# Autodesk Inventor assembly: GripperBaseOnly
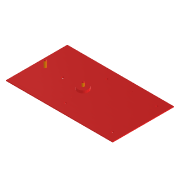
[picture p0: Inventor's stored thumbnail of the model, 180x180]
Saved by Autodesk Inventor 2021 (Build 250183000, 183)
## iProperties
Created: 2022-10-24
Part Number: GripperBaseOnly
Document SubType Name: Assembly
Designer: brian
Author: brian
## Documents named in this file (2)
- G:\Mi unidad\Universidad\Control\Robotica\Laboratorio\Proyecto\Archivos SAT\GripperBasePlace.iam
- G:\Mi unidad\Universidad\Control\Robotica\Laboratorio\Proyecto\GriperBase2.ipt
## Components (1 placed, 1 different names)
1. GriperBase2:1 — Mate:1, Tangent:1, Tangent:2
## Relationships (3: Tangent 2, Mate 1)
- Mate:1: GriperBase2:1
- Tangent:1: GriperBase2:1
- Tangent:2: GriperBase2:1
